# Autodesk Inventor assembly: handle
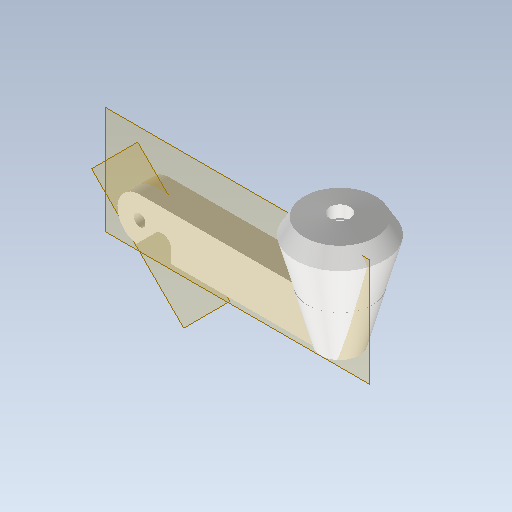
[picture p0: Inventor's stored thumbnail of the model, 512x512]
Saved by Autodesk Inventor 2021 (Build 250183000, 183)
## iProperties
Created: 2021-06-09
Part Number: handle
Document SubType Name: Assembly
Designer: teh18
Author: teh18
## Documents named in this file (3)
- C:\Users\teh18\OneDrive\BVE Controller\r68-bve-mascon\handle\handle.iam
- C:\Users\teh18\OneDrive\BVE Controller\r68-bve-mascon\handle\metal.ipt
- C:\Users\teh18\OneDrive\BVE Controller\r68-bve-mascon\handle\free rotating sheath.ipt
## Components (2 placed, 2 different names)
1. metal:1 — Mate:3, Mate:4
2. free rotating sheath:2 — Mate:3, Mate:4
## Relationships (2: Mate 2)
- Mate:3: metal:1 ↔ free rotating sheath:2
- Mate:4: metal:1 ↔ free rotating sheath:2
